# Autodesk Inventor assembly: Assembly_Cana
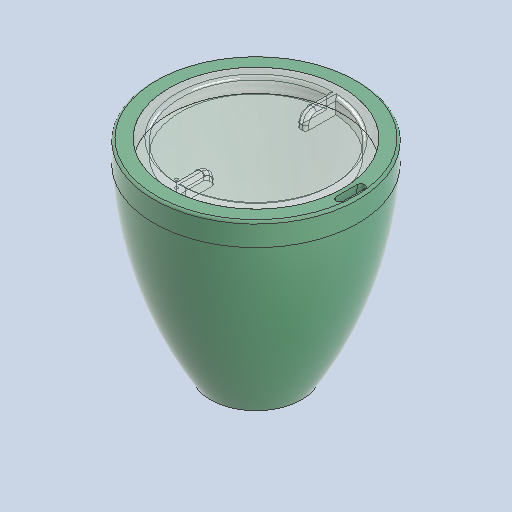
[picture p0: Inventor's stored thumbnail of the model, 512x512]
Saved by Autodesk Inventor 2025.2 (Build 292293000, 293)
## iProperties
Created: 2024-05-14
Part Number: Assembly_Cana
Document SubType Name: Assembly
Designer: mirun
Author: mirun
## Documents named in this file (3)
- C:\Users\mirewn\OneDrive - Universitatea Politehnica Bucuresti\AA- Projects\Cana_estetica\Assembly_Mug.iam
- C:\Users\mirewn\OneDrive - Universitatea Politehnica Bucuresti\AA- Projects\Cana_estetica\Mug.ipt
- C:\Users\mirewn\OneDrive - Universitatea Politehnica Bucuresti\AA- Projects\Cana_estetica\Lid.ipt
## Components (2 placed, 2 different names)
1. Mug:1 — Mate:1, Flush:1
2. Lid:1 — Mate:1, Flush:1
## Relationships (2: Mate 1, Flush 1)
- Mate:1: Mug:1 ↔ Lid:1
- Flush:1: Mug:1 ↔ Lid:1
